# Autodesk Inventor assembly: Ensamble
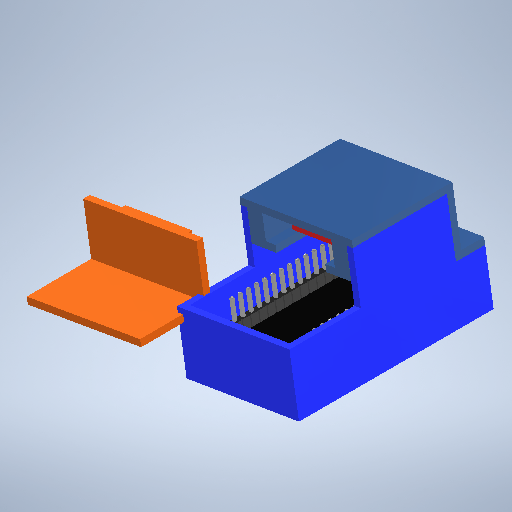
[picture p0: Inventor's stored thumbnail of the model, 512x512]
Saved by Autodesk Inventor 2025.1 (Build 291241020, 241B)
## iProperties
Created: 2024-08-30
Part Number: Ensamble
Document SubType Name: Assembly
Designer: andre
Author: andre
## Documents named in this file (7)
- C:\Users\andre\OneDrive_Personal\OneDrive\UCR\TCU\Diseño\Ensamble.iam
- C:\Users\andre\OneDrive_Personal\OneDrive\UCR\TCU\Diseño\Carcaza.ipt
- C:\Users\andre\OneDrive_Personal\OneDrive\UCR\TCU\Diseño\ESP32_DevBoard.ipt
- C:\Users\andre\OneDrive_Personal\OneDrive\UCR\TCU\Diseño\Circuit.ipt
- C:\Users\andre\OneDrive_Personal\OneDrive\UCR\TCU\Diseño\TapaCarcaza.ipt
- C:\Users\andre\OneDrive_Personal\OneDrive\UCR\TCU\Diseño\TapaTrasera.ipt
- C:\Users\andre\OneDrive_Personal\OneDrive\UCR\TCU\Diseño\CableFemale.ipt
## Components (8 placed, 6 different names)
1. Carcaza:1 — Mate:21, Mate:22, Mate:23, Mate:24, Mate:25, Mate:26
2. ESP32_DevBoard:1 — Mate:14, Mate:15, Mate:16, Mate:17, Mate:18, Mate:19, Mate:20, Mate:21, Mate:22, Mate:25
3. Circuit:1 — Mate:5, Mate:13
4. TapaCarcaza:1 — Mate:5, Mate:13, Mate:23, Mate:24, Mate:26
5. TapaTrasera:1
6. CableFemale:1 — Mate:16, Mate:17, Mate:18
7. CableFemale:2 — Mate:19, Mate:20
8. CableFemale:3 — Mate:14, Mate:15
## Relationships (15: Mate 15)
- Mate:5: Circuit:1 ↔ TapaCarcaza:1
- Mate:13 (1.25 mm): Circuit:1 ↔ TapaCarcaza:1
- Mate:14: ESP32_DevBoard:1 ↔ CableFemale:3
- Mate:15: ESP32_DevBoard:1 ↔ CableFemale:3
- Mate:16: ESP32_DevBoard:1 ↔ CableFemale:1
- Mate:17: ESP32_DevBoard:1 ↔ CableFemale:1
- Mate:18: ESP32_DevBoard:1 ↔ CableFemale:1
- Mate:19: ESP32_DevBoard:1 ↔ CableFemale:2
- Mate:20: ESP32_DevBoard:1 ↔ CableFemale:2
- Mate:21: Carcaza:1 ↔ ESP32_DevBoard:1
- Mate:22: Carcaza:1 ↔ ESP32_DevBoard:1
- Mate:23: Carcaza:1 ↔ TapaCarcaza:1
- Mate:24: Carcaza:1 ↔ TapaCarcaza:1
- Mate:25 (2.5 mm): Carcaza:1 ↔ ESP32_DevBoard:1
- Mate:26: Carcaza:1 ↔ TapaCarcaza:1
## Named parameters: w = 2 mm
